# Autodesk Inventor assembly: base wheel
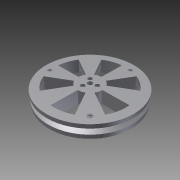
[picture p0: Inventor's stored thumbnail of the model, 180x180]
Saved by Autodesk Inventor 2011 (Build 150239000, 239)
## iProperties
Created: 2010-04-18
Part Number: base wheel
Document SubType Name: Assembly
Designer: lucio
Mass: 196.688 g
Surface Area: 712.661 cm^2
Volume: 199.418 cm^3
Density: 0.98631 g/cm^3
Author: lucio
## Documents named in this file (4)
- C:\Users\lucio\Documents\Inventor\caterpillar\base wheel.iam
- C:\Users\lucio\Documents\Inventor\caterpillar\wheel.ipt
- C:\Users\lucio\Documents\Inventor\Content Center Files\R2011\en-US\ANSI B18.3.1M(5)\ANSI B18.3.1M - M4x0.7 x 16(3).ipt
- C:\Users\lucio\Documents\Inventor\Content Center Files\R2011\en-US\ANSI B 18.2.4.1 M(1)\ANSI B 18.2.4.1 M - M4 x 0.7Style 2.ipt
## Components (8 placed, 3 different names)
1. wheel:1 — Mate:1, Mate:2, Mate:3, Insert:12
2. wheel:2 — Insert:9, Insert:10, Insert:11, Mate:1
3. Drilled Forged Hexagon Socket Head Cap Screw - 6 Holes - Metric M4x0.7 x 16:1 — Insert:9
4. Drilled Forged Hexagon Socket Head Cap Screw - 6 Holes - Metric M4x0.7 x 16:2 — Insert:10, Mate:3, Insert:14
5. Drilled Forged Hexagon Socket Head Cap Screw - 6 Holes - Metric M4x0.7 x 16:4 — Insert:11, Mate:2, Insert:13
6. Hex Nut Metric M4 x 0.7:1 — Insert:14
7. Hex Nut Metric M4 x 0.7:2 — Insert:13
8. Hex Nut Metric M4 x 0.7:3 — Insert:12
## Relationships (9: Insert 6, Mate 3)
- Insert:9: wheel:2 ↔ Drilled Forged Hexagon Socket Head Cap Screw - 6 Holes - Metric M4x0.7 x 16:1
- Insert:10: wheel:2 ↔ Drilled Forged Hexagon Socket Head Cap Screw - 6 Holes - Metric M4x0.7 x 16:2
- Insert:11: wheel:2 ↔ Drilled Forged Hexagon Socket Head Cap Screw - 6 Holes - Metric M4x0.7 x 16:4
- Mate:1: wheel:1 ↔ wheel:2
- Mate:2: wheel:1 ↔ Drilled Forged Hexagon Socket Head Cap Screw - 6 Holes - Metric M4x0.7 x 16:4
- Mate:3: wheel:1 ↔ Drilled Forged Hexagon Socket Head Cap Screw - 6 Holes - Metric M4x0.7 x 16:2
- Insert:12: wheel:1 ↔ Hex Nut Metric M4 x 0.7:3
- Insert:13: Drilled Forged Hexagon Socket Head Cap Screw - 6 Holes - Metric M4x0.7 x 16:4 ↔ Hex Nut Metric M4 x 0.7:2
- Insert:14: Drilled Forged Hexagon Socket Head Cap Screw - 6 Holes - Metric M4x0.7 x 16:2 ↔ Hex Nut Metric M4 x 0.7:1
